# Autodesk Inventor assembly: idler pully for pickerupthingy
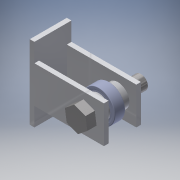
[picture p0: Inventor's stored thumbnail of the model, 180x180]
Saved by Autodesk Inventor 2016 (Build 200138000, 138)
## iProperties
Created: 2016-02-24
Part Number: idler pully for pickerupthingy
Document SubType Name: Assembly
Designer: gus
Author: gus
## Documents named in this file (5)
- \\Mac\Home\Desktop\1510-stronghold-CAD-master\idler pully for pickerupthingy\idler pully for pickerupthingy.iam
- \\Mac\Home\Desktop\1510-stronghold-CAD-master\idler pully for pickerupthingy\base.ipt
- \\Mac\Home\Desktop\1510-stronghold-CAD-master\idler pully for pickerupthingy\bolt.ipt
- \\Mac\Home\Desktop\1510-stronghold-CAD-master\idler pully for pickerupthingy\217-3239-STEP.ipt
- \\Mac\Home\Desktop\1510-stronghold-CAD-master\idler pully for pickerupthingy\spacer.ipt
## Components (5 placed, 4 different names)
1. base:1 — Flush:1, Mate:1, Mate:7
2. bolt:1 — Flush:1, Mate:1, Mate:2, Mate:6
3. 217-3239-STEP:1 — Mate:2, Mate:3, Mate:4, Mate:5
4. spacer:1 — Mate:5, Mate:6, Mate:7
5. spacer:2 — Mate:3, Mate:4
## Relationships (8: Mate 7, Flush 1)
- Flush:1: base:1 ↔ bolt:1
- Mate:1: base:1 ↔ bolt:1
- Mate:2: bolt:1 ↔ 217-3239-STEP:1
- Mate:3: 217-3239-STEP:1 ↔ spacer:2
- Mate:4: 217-3239-STEP:1 ↔ spacer:2
- Mate:5: 217-3239-STEP:1 ↔ spacer:1
- Mate:6: bolt:1 ↔ spacer:1
- Mate:7: base:1 ↔ spacer:1
